# Autodesk Inventor assembly: pullboxFiber
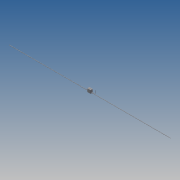
[picture p0: Inventor's stored thumbnail of the model, 180x180]
Saved by Autodesk Inventor 2014 SP1 (Build 180222100, 222)
## iProperties
Created: 2014-12-12
Part Number: pullboxFiber
Document SubType Name: Assembly
Designer: Dave
Author: Dave
## Documents named in this file (7)
- C:\Users\Dave\Desktop\hera-cad\Node\pullboxFiber.iam
- C:\Users\Dave\Desktop\hera-cad\Node\pullboxFiber.ipt
- C:\Users\Dave\Desktop\hera-cad\Node\pipe_100mm_1.5m.ipt
- C:\Users\Dave\Desktop\hera-cad\Node\pipe_50mm_0.5m.ipt
- C:\Users\Dave\Desktop\hera-cad\Node\sweep_50mm.ipt
- C:\Users\Dave\Desktop\hera-cad\Node\pullboxFiberLid.ipt
- C:\Users\Dave\Desktop\hera-cad\Node\pipe_100mm_Long.ipt
## Components (9 placed, 6 different names)
1. pullboxFiber:2 — Insert:1, Insert:2, Insert:3, Angle:1, Flush:1, Flush:2, Mate:1
2. pipe_50mm_0.5m:1 — Insert:5, Angle:1
3. pipe_50mm_0.5m:2 — Insert:3, Insert:4
4. sweep_50mm:1 — Insert:4, Insert:5
5. pipe_100mm_1.5m:1 — Insert:1, Insert:6
6. pipe_100mm_1.5m:2 — Insert:2, Insert:7
7. pullboxFiberLid:1 — Flush:1, Flush:2, Mate:1
8. pipe_100mm_Long:1 — Insert:7
9. pipe_100mm_Long:2 — Insert:6
## Relationships (11: Insert 7, Flush 2, Angle 1, Mate 1)
- Insert:1: pullboxFiber:2 ↔ pipe_100mm_1.5m:1
- Insert:2: pullboxFiber:2 ↔ pipe_100mm_1.5m:2
- Insert:3: pullboxFiber:2 ↔ pipe_50mm_0.5m:2
- Insert:4: pipe_50mm_0.5m:2 ↔ sweep_50mm:1
- Insert:5 (-101.6 mm): pipe_50mm_0.5m:1 ↔ sweep_50mm:1
- Angle:1 (180 deg): pullboxFiber:2 ↔ pipe_50mm_0.5m:1
- Flush:1: pullboxFiber:2 ↔ pullboxFiberLid:1
- Flush:2: pullboxFiber:2 ↔ pullboxFiberLid:1
- Mate:1 (5.08 mm): pullboxFiber:2 ↔ pullboxFiberLid:1
- Insert:6: pipe_100mm_1.5m:1 ↔ pipe_100mm_Long:2
- Insert:7: pipe_100mm_1.5m:2 ↔ pipe_100mm_Long:1
